# Autodesk Inventor assembly: ES117_MBody
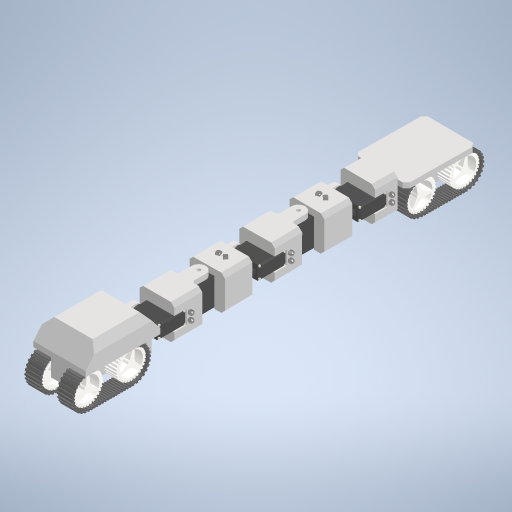
[picture p0: Inventor's stored thumbnail of the model, 512x512]
Saved by Autodesk Inventor 2024 (Build 280153000, 153)
## iProperties
Created: 2023-06-04
Part Number: ES117_MBody
Document SubType Name: Assembly
Designer: vilas
Author: vilas
## Documents named in this file (10)
- D:\Parth Folder\ES117\3D Model\Prototype 1\MBody.iam
- D:\Parth Folder\ES117\3D Model\Prototype 1\MP1.ipt
- D:\Parth Folder\ES117\3D Model\Prototype 1\MG995.ipt
- D:\Parth Folder\ES117\3D Model\Prototype 1\MP2.ipt
- D:\Parth Folder\ES117\3D Model\Prototype 1\Bolt.ipt
- D:\Parth Folder\ES117\3D Model\Prototype 1\Nut.ipt
- D:\Parth Folder\ES117\3D Model\Prototype 1\Head.ipt
- D:\Parth Folder\ES117\3D Model\Prototype 1\Tail.ipt
- D:\Parth Folder\ES117\3D Model\Prototype 1\Wheel(1).ipt
- D:\Parth Folder\ES117\3D Model\Prototype 1\Track(1).ipt
## Components (43 placed, 9 different names)
1. MP1:1 — Mate:1, Mate:2, Mate:3, Mate:7, Flush:1, Mate:8, Mate:9, Mate:10, Mate:11, Mate:16, Mate:18
2. MG995:1 — Mate:1, Mate:2, Mate:3, Mate:50, Mate:51
3. MP2:1 — Mate:4, Mate:5, Mate:6, Flush:1, Mate:12, Mate:13, Mate:14, Mate:15, Mate:20, Mate:21, Mate:35, Flush:2
4. MG995:2 — Mate:4, Mate:5, Mate:6, Mate:7
5. Bolt:1 — Mate:10, Mate:11, Mate:19
6. Bolt:2 — Mate:8, Mate:9, Mate:17
7. Bolt:3 — Mate:12, Mate:13, Mate:23
8. Bolt:4 — Mate:14, Mate:15, Mate:22
9. Nut:1 — Mate:16, Mate:17
10. Nut:2 — Mate:18, Mate:19
11. Nut:3 — Mate:20, Mate:22
12. Nut:4 — Mate:21, Mate:23
13. MP1:2 — Flush:2, Mate:47, Flush:3
14. MG995:3 — Mate:35
15. Bolt:5
16. Bolt:6
17. Nut:5
18. Nut:6
19. MP2:2 — Flush:3, Mate:48, Mate:49
20. MG995:4 — Mate:47
21. Bolt:7
22. Bolt:8
23. Nut:7
24. Nut:8
25. MG995:5 — Mate:48, Mate:49, Mate:52, Mate:53, Mate:54
26. Head:1 — Mate:50, Mate:51, Mate:63, Mate:64, Mate:65, Mate:66, Mate:67, Mate:68, Mate:69, Mate:70, Mate:79, Mate:80
27. Tail:1 — Mate:52, Mate:53, Mate:54, Mate:55, Mate:56, Mate:57, Mate:58, Mate:61, Mate:62, Mate:71, Mate:72, Mate:73, Mate:74, Mate:75, Mate:76, Mate:77, Mate:78, Mate:81, Mate:82
28. Bolt:9 — Mate:55, Mate:56, Mate:60
29. Bolt:10 — Mate:57, Mate:58, Mate:59
30. Nut:9 — Mate:59, Mate:62
31. Nut:10 — Mate:60, Mate:61
32. Wheel(1):1 — Mate:69, Mate:70
33. Wheel(1):2 — Mate:67, Mate:68
34. Wheel(1):3 — Mate:63, Mate:64
35. Wheel(1):4 — Mate:65, Mate:66
36. Wheel(1):5 — Mate:73, Mate:74
37. Wheel(1):6 — Mate:71, Mate:72
38. Wheel(1):7 — Mate:76, Mate:78
39. Wheel(1):8 — Mate:75, Mate:77
40. Track(1):1 — Mate:79
41. Track(1):2 — Mate:80
42. Track(1):3 — Mate:81
43. Track(1):4 — Mate:82
## Relationships (85: Mate 82, Flush 3)
- Mate:1: MP1:1 ↔ MG995:1
- Mate:2: MP1:1 ↔ MG995:1
- Mate:3: MP1:1 ↔ MG995:1
- Mate:4: MP2:1 ↔ MG995:2
- Mate:5: MP2:1 ↔ MG995:2
- Mate:6: MP2:1 ↔ MG995:2
- Mate:7: MP1:1 ↔ MG995:2
- Flush:1: MP1:1 ↔ MP2:1
- Mate:8: MP1:1 ↔ Bolt:2
- Mate:9: MP1:1 ↔ Bolt:2
- Mate:10: MP1:1 ↔ Bolt:1
- Mate:11: MP1:1 ↔ Bolt:1
- Mate:12: MP2:1 ↔ Bolt:3
- Mate:13: MP2:1 ↔ Bolt:3
- Mate:14: MP2:1 ↔ Bolt:4
- Mate:15: MP2:1 ↔ Bolt:4
- Mate:16: MP1:1 ↔ Nut:1
- Mate:17: Bolt:2 ↔ Nut:1
- Mate:18: MP1:1 ↔ Nut:2
- Mate:19: Bolt:1 ↔ Nut:2
- Mate:20: MP2:1 ↔ Nut:3
- Mate:21: MP2:1 ↔ Nut:4
- Mate:22: Bolt:4 ↔ Nut:3
- Mate:23: Bolt:3 ↔ Nut:4
- [Mate]: MP1:2 ↔ MG995:3
- [Mate]: MP1:2 ↔ MG995:3
- [Mate]: MP1:2 ↔ MG995:3
- [Mate]: MP1:2 ↔ Bolt:6
- [Mate]: MP1:2 ↔ Bolt:6
- [Mate]: MP1:2 ↔ Bolt:5
- [Mate]: MP1:2 ↔ Bolt:5
- [Mate]: MP1:2 ↔ Nut:5
- [Mate]: Bolt:6 ↔ Nut:5
- [Mate]: MP1:2 ↔ Nut:6
- [Mate]: Bolt:5 ↔ Nut:6
- Mate:35: MP2:1 ↔ MG995:3
- Flush:2: MP2:1 ↔ MP1:2
- [Mate]: MP2:2 ↔ MG995:4
- [Mate]: MP2:2 ↔ MG995:4
- [Mate]: MP2:2 ↔ MG995:4
- [Mate]: MP2:2 ↔ Bolt:7
- [Mate]: MP2:2 ↔ Bolt:7
- [Mate]: MP2:2 ↔ Bolt:8
- [Mate]: MP2:2 ↔ Bolt:8
- [Mate]: MP2:2 ↔ Nut:7
- [Mate]: MP2:2 ↔ Nut:8
- [Mate]: Bolt:8 ↔ Nut:7
- [Mate]: Bolt:7 ↔ Nut:8
- Mate:47: MP1:2 ↔ MG995:4
- Flush:3: MP1:2 ↔ MP2:2
- Mate:48: MP2:2 ↔ MG995:5
- Mate:49: MP2:2 ↔ MG995:5
- Mate:50: MG995:1 ↔ Head:1
- Mate:51: MG995:1 ↔ Head:1
- Mate:52: MG995:5 ↔ Tail:1
- Mate:53: MG995:5 ↔ Tail:1
- Mate:54: MG995:5 ↔ Tail:1
- Mate:55: Tail:1 ↔ Bolt:9
- Mate:56: Tail:1 ↔ Bolt:9
- Mate:57: Tail:1 ↔ Bolt:10
- Mate:58: Tail:1 ↔ Bolt:10
- Mate:59: Bolt:10 ↔ Nut:9
- Mate:60: Bolt:9 ↔ Nut:10
- Mate:61: Tail:1 ↔ Nut:10
- Mate:62: Tail:1 ↔ Nut:9
- Mate:63: Head:1 ↔ Wheel(1):3
- Mate:64: Head:1 ↔ Wheel(1):3
- Mate:65: Head:1 ↔ Wheel(1):4
- Mate:66: Head:1 ↔ Wheel(1):4
- Mate:67: Head:1 ↔ Wheel(1):2
- Mate:68: Head:1 ↔ Wheel(1):2
- Mate:69: Head:1 ↔ Wheel(1):1
- Mate:70: Head:1 ↔ Wheel(1):1
- Mate:71: Tail:1 ↔ Wheel(1):6
- Mate:72: Tail:1 ↔ Wheel(1):6
- Mate:73: Tail:1 ↔ Wheel(1):5
- Mate:74: Tail:1 ↔ Wheel(1):5
- Mate:75: Tail:1 ↔ Wheel(1):8
- Mate:76: Tail:1 ↔ Wheel(1):7
- Mate:77: Tail:1 ↔ Wheel(1):8
- Mate:78: Tail:1 ↔ Wheel(1):7
- Mate:79: Head:1 ↔ Track(1):1
- Mate:80: Head:1 ↔ Track(1):2
- Mate:81: Tail:1 ↔ Track(1):3
- Mate:82: Tail:1 ↔ Track(1):4
## Named parameters: d34_d3 = 0 mm, d35_d4 = 0 mm, d36_d5 = 0 mm, d37_d18 = 0 mm, d38_d19 = 0 mm, d39_d20 = 0 mm, d40_d21 = 0 mm, d41_d26 = 0 mm, d42_d27 = 0 mm, d43_d28 = 0 mm, d44_d29 = 0 mm, d47_d12 = 0 mm, d48_d13 = 0 mm, d49_d14 = 0 mm, d50_d22 = 0 mm, d51_d23 = 0 mm, d52_d24 = 0 mm, d53_d25 = 0 mm, d54_d30 = 0 mm, d55_d31 = 0 mm, d56_d32 = 0 mm, d57_d33 = 0 mm
